# Autodesk Inventor assembly: Assembly1
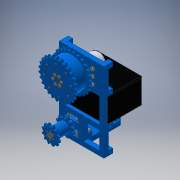
[picture p0: Inventor's stored thumbnail of the model, 180x180]
Saved by Autodesk Inventor 2016 (Build 200138000, 138)
## iProperties
Created: 2016-06-04
Part Number: Assembly1
Document SubType Name: Assembly
Designer: hesaon
Author: hesaon
## Documents named in this file (24)
- C:\Users\hesaon\Documents\Killer-Bot-2016\AutodeskWorkspace\robotparts revision 2\Assembly1.iam
- C:\Users\hesaon\Documents\Killer-Bot-2016\AutodeskWorkspace\robotparts revision 2\sideFrame.ipt
- C:\Users\hesaon\Documents\Killer-Bot-2016\AutodeskWorkspace\robotparts revision 2\motorHolder57mmVer2.ipt
- C:\Users\hesaon\Documents\Killer-Bot-2016\AutodeskWorkspace\robotparts revision 2\nut4mm.ipt
- C:\Users\hesaon\Documents\Killer-Bot-2016\AutodeskWorkspace\robotparts revision 2\screw18x4mm.ipt
- C:\Users\hesaon\Documents\Killer-Bot-2016\AutodeskWorkspace\robotparts revision 2\washer4mm.ipt
- C:\Users\hesaon\Documents\Killer-Bot-2016\AutodeskWorkspace\robotparts revision 2\37D mm metal gearmotor.ipt
- C:\Users\hesaon\Documents\Killer-Bot-2016\AutodeskWorkspace\robotparts revision 2\washer3mm.ipt
- C:\Users\hesaon\Documents\Killer-Bot-2016\AutodeskWorkspace\robotparts revision 2\screw12x3mm.ipt
- C:\Users\hesaon\Documents\Killer-Bot-2016\AutodeskWorkspace\robotparts revision 2\mountingHub6mm.ipt
- C:\Users\hesaon\Documents\Killer-Bot-2016\AutodeskWorkspace\robotparts revision 2\outerBigSprocket2.ipt
- C:\Users\hesaon\Documents\Killer-Bot-2016\AutodeskWorkspace\robotparts revision 2\sprocketsHolder.ipt
- C:\Users\hesaon\Documents\Killer-Bot-2016\AutodeskWorkspace\robotparts revision 2\BigSprocket2.ipt
- C:\Users\hesaon\Documents\Killer-Bot-2016\AutodeskWorkspace\robotparts revision 2\screwKa22x16.ipt
- C:\Users\hesaon\Documents\Killer-Bot-2016\AutodeskWorkspace\robotparts revision 2\battery.ipt
- C:\Users\hesaon\Documents\Killer-Bot-2016\AutodeskWorkspace\robotparts revision 2\backFrame.ipt
- C:\Users\hesaon\Documents\Killer-Bot-2016\AutodeskWorkspace\robotparts revision 2\screw27x4mm.ipt
- C:\Users\hesaon\Documents\Killer-Bot-2016\AutodeskWorkspace\robotparts revision 2\pin5x60.ipt
- C:\Users\hesaon\Documents\Killer-Bot-2016\AutodeskWorkspace\robotparts revision 2\smallSprocketFixture.ipt
- C:\Users\hesaon\Documents\Killer-Bot-2016\AutodeskWorkspace\robotparts revision 2\nut6mm.ipt
- C:\Users\hesaon\Documents\Killer-Bot-2016\AutodeskWorkspace\robotparts revision 2\washer6mm.ipt
- C:\Users\hesaon\Documents\Killer-Bot-2016\AutodeskWorkspace\robotparts revision 2\smallSprocketDistance.ipt
- C:\Users\hesaon\Documents\Killer-Bot-2016\AutodeskWorkspace\robotparts revision 2\smallSprocket.ipt
- C:\Users\hesaon\Documents\Killer-Bot-2016\AutodeskWorkspace\robotparts revision 2\smallSprocketHolder.ipt
## Components (105 placed, 22 different names)
1. sideFrame:1 — Insert:1, Insert:2, Insert:3, Insert:4, Insert:5, Insert:6, Insert:7, Insert:8, Flush:1, Mate:1, Mate:2, Insert:80, Insert:81, Insert:86, Insert:87, Insert:90, Insert:91
2. motorHolder57mmVer2:1 — Insert:1, Insert:2, Insert:9, Insert:10, Insert:11, Insert:12, Insert:13, Insert:14, Insert:27, Insert:28, Insert:29, Insert:30, Insert:31, Insert:32, Insert:33, Insert:34
3. nut4mm:1 — Insert:26
4. nut4mm:2 — Insert:21
5. nut4mm:3 — Insert:22
6. nut4mm:4 — Insert:23
7. nut4mm:5 — Insert:24
8. nut4mm:6 — Insert:25
9. screw18x4mm:1 — Insert:17
10. screw18x4mm:2 — Insert:19
11. screw18x4mm:3 — Insert:16
12. screw18x4mm:4 — Insert:15
13. screw18x4mm:5 — Insert:18
14. screw18x4mm:6 — Insert:20
15. washer4mm:1 — Insert:5, Insert:21
16. washer4mm:2 — Insert:8, Insert:24
17. washer4mm:3 — Insert:10, Insert:17
18. washer4mm:4 — Insert:9, Insert:15
19. washer4mm:5 — Insert:11, Insert:18
20. washer4mm:6 — Insert:12, Insert:19
21. washer4mm:7 — Insert:7, Insert:26
22. washer4mm:8 — Insert:13, Insert:16
23. washer4mm:9 — Insert:14, Insert:20
24. washer4mm:10 — Insert:4, Insert:23
25. washer4mm:11 — Insert:3, Insert:22
26. washer4mm:12 — Insert:6, Insert:25
27. 37D mm metal gearmotor:1 — Insert:27, Insert:28, Insert:41
28. washer3mm:1 — Insert:29, Insert:37
29. washer3mm:2 — Insert:30, Insert:36
30. washer3mm:3 — Insert:32, Insert:40
31. washer3mm:4 — Insert:31, Insert:35
32. washer3mm:5 — Insert:33, Insert:39
33. washer3mm:6 — Insert:34, Insert:38
34. screw12x3mm:1 — Insert:38
35. screw12x3mm:2 — Insert:35
36. screw12x3mm:3 — Insert:36
37. screw12x3mm:4 — Insert:37
38. screw12x3mm:5 — Insert:40
39. screw12x3mm:6 — Insert:39
40. mountingHub6mm:1 — Insert:41, Insert:42, Insert:43
41. Outer big sprocket:1 — Insert:42, Insert:43, Insert:44, Insert:45, Insert:48, Insert:49, Insert:50, Insert:51, Insert:52, Insert:53, Insert:54, Insert:55, Insert:64, Insert:65, Insert:66, Insert:67, Insert:68, Insert:69
42. sprocketsHolder:1 — Insert:44, Insert:45, Insert:46, Insert:47
43. Roller Chain Sprocket1:1 — Insert:46, Insert:47, Insert:56, Insert:57, Insert:58, Insert:59, Insert:60, Insert:61, Insert:62, Insert:63
44. screwKa22x16:1 — Insert:56
45. screwKa22x16:2 — Insert:57
46. screwKa22x16:3 — Insert:58
47. screwKa22x16:4 — Insert:59
48. screwKa22x16:5 — Insert:60
49. screwKa22x16:6 — Insert:61
50. screwKa22x16:7 — Insert:63
51. screwKa22x16:8 — Insert:62
52. screwKa22x16:9 — Insert:48
53. screwKa22x16:10 — Insert:49
54. screwKa22x16:11 — Insert:50
55. screwKa22x16:12 — Insert:51
56. screwKa22x16:13 — Insert:52
57. screwKa22x16:14 — Insert:53
58. screwKa22x16:15 — Insert:54
59. screwKa22x16:16 — Insert:55
60. washer3mm:7 — Insert:64, Insert:70
61. washer3mm:8 — Insert:65, Insert:74
62. washer3mm:9 — Insert:66, Insert:75
63. washer3mm:10 — Insert:67, Insert:73
64. washer3mm:11 — Insert:68, Insert:72
65. washer3mm:12 — Insert:69, Insert:71
66. screw12x3mm:7 — Insert:70
67. screw12x3mm:8 — Insert:71
68. screw12x3mm:9 — Insert:72
69. screw12x3mm:10 — Insert:73
70. screw12x3mm:11 — Insert:74
71. screw12x3mm:12 — Insert:75
72. battery:1 — Flush:1, Mate:1, Mate:2
73. backFrame:1 — Insert:86, Insert:87, Insert:88, Insert:89
74. nut4mm:7 — Insert:85
75. nut4mm:8 — Insert:84
76. washer4mm:13 — Insert:82, Insert:89
77. washer4mm:14 — Insert:83, Insert:88
78. washer4mm:15 — Insert:80, Insert:85
79. washer4mm:16 — Insert:81, Insert:84
80. screw27x4mm:1 — Insert:83
81. screw27x4mm:2 — Insert:82
82. pin5x60:1 — Insert:91, Cylindrical:2
83. pin5x60:2 — Insert:90, Cylindrical:1
84. smallSprocketFixture:1 — Cylindrical:1, Cylindrical:2, Insert:92, Angle:1, Insert:94
85. nut6mm:1 — Insert:92, Angle:1, Insert:93
86. washer6mm:1 — Insert:93, Insert:95
87. washer6mm:2 — Insert:94
88. smallSprocketDistance:1 — Insert:95, Insert:96
89. washer6mm:3 — Insert:96, Insert:97
90. Roller Chain Sprocket1:2 — Insert:100, Insert:101, Insert:102, Insert:103, Insert:104, Insert:105, Insert:106, Insert:107, Insert:114
91. Roller Chain Sprocket1:3 — Insert:97, Insert:98, Insert:99, Insert:108, Insert:109, Insert:110, Insert:111, Insert:112, Insert:113
92. smallSprocketHolder:1 — Insert:98, Insert:99, Insert:100, Insert:101
93. screwKa22x16:17 — Insert:111
94. screwKa22x16:18 — Insert:104
95. screwKa22x16:19 — Insert:105
96. screwKa22x16:20 — Insert:106
97. screwKa22x16:21 — Insert:107
98. screwKa22x16:22 — Insert:109
99. screwKa22x16:23 — Insert:110
100. screwKa22x16:24 — Insert:112
101. screwKa22x16:25 — Insert:113
102. screwKa22x16:26 — Insert:108
103. screwKa22x16:27 — Insert:103
104. screwKa22x16:28 — Insert:102
105. washer6mm:4 — Insert:114
## Relationships (116: Insert 110, Mate 2, CylindricalJoint 2, Flush 1, Angle 1)
- Insert:1: sideFrame:1 ↔ motorHolder57mmVer2:1
- Insert:2: sideFrame:1 ↔ motorHolder57mmVer2:1
- Insert:3: sideFrame:1 ↔ washer4mm:11
- Insert:4: sideFrame:1 ↔ washer4mm:10
- Insert:5: sideFrame:1 ↔ washer4mm:1
- Insert:6: sideFrame:1 ↔ washer4mm:12
- Insert:7: sideFrame:1 ↔ washer4mm:7
- Insert:8: sideFrame:1 ↔ washer4mm:2
- Insert:9: motorHolder57mmVer2:1 ↔ washer4mm:4
- Insert:10: motorHolder57mmVer2:1 ↔ washer4mm:3
- Insert:11: motorHolder57mmVer2:1 ↔ washer4mm:5
- Insert:12: motorHolder57mmVer2:1 ↔ washer4mm:6
- Insert:13: motorHolder57mmVer2:1 ↔ washer4mm:8
- Insert:14: motorHolder57mmVer2:1 ↔ washer4mm:9
- Insert:15: screw18x4mm:4 ↔ washer4mm:4
- Insert:16: screw18x4mm:3 ↔ washer4mm:8
- Insert:17: screw18x4mm:1 ↔ washer4mm:3
- Insert:18: screw18x4mm:5 ↔ washer4mm:5
- Insert:19: screw18x4mm:2 ↔ washer4mm:6
- Insert:20: screw18x4mm:6 ↔ washer4mm:9
- Insert:21: nut4mm:2 ↔ washer4mm:1
- Insert:22: nut4mm:3 ↔ washer4mm:11
- Insert:23: nut4mm:4 ↔ washer4mm:10
- Insert:24: nut4mm:5 ↔ washer4mm:2
- Insert:25: nut4mm:6 ↔ washer4mm:12
- Insert:26: nut4mm:1 ↔ washer4mm:7
- Insert:27: motorHolder57mmVer2:1 ↔ 37D mm metal gearmotor:1
- Insert:28: motorHolder57mmVer2:1 ↔ 37D mm metal gearmotor:1
- Insert:29: motorHolder57mmVer2:1 ↔ washer3mm:1
- Insert:30: motorHolder57mmVer2:1 ↔ washer3mm:2
- Insert:31: motorHolder57mmVer2:1 ↔ washer3mm:4
- Insert:32: motorHolder57mmVer2:1 ↔ washer3mm:3
- Insert:33: motorHolder57mmVer2:1 ↔ washer3mm:5
- Insert:34: motorHolder57mmVer2:1 ↔ washer3mm:6
- Insert:35: washer3mm:4 ↔ screw12x3mm:2
- Insert:36: washer3mm:2 ↔ screw12x3mm:3
- Insert:37: washer3mm:1 ↔ screw12x3mm:4
- Insert:38: washer3mm:6 ↔ screw12x3mm:1
- Insert:39: washer3mm:5 ↔ screw12x3mm:6
- Insert:40: washer3mm:3 ↔ screw12x3mm:5
- Insert:41: 37D mm metal gearmotor:1 ↔ mountingHub6mm:1
- Insert:42: mountingHub6mm:1 ↔ Outer big sprocket:1
- Insert:43: mountingHub6mm:1 ↔ Outer big sprocket:1
- Insert:44: Outer big sprocket:1 ↔ sprocketsHolder:1
- Insert:45: Outer big sprocket:1 ↔ sprocketsHolder:1
- Insert:46: sprocketsHolder:1 ↔ Roller Chain Sprocket1:1
- Insert:47: sprocketsHolder:1 ↔ Roller Chain Sprocket1:1
- Insert:48: Outer big sprocket:1 ↔ screwKa22x16:9
- Insert:49: Outer big sprocket:1 ↔ screwKa22x16:10
- Insert:50: Outer big sprocket:1 ↔ screwKa22x16:11
- Insert:51: Outer big sprocket:1 ↔ screwKa22x16:12
- Insert:52: Outer big sprocket:1 ↔ screwKa22x16:13
- Insert:53: Outer big sprocket:1 ↔ screwKa22x16:14
- Insert:54: Outer big sprocket:1 ↔ screwKa22x16:15
- Insert:55: Outer big sprocket:1 ↔ screwKa22x16:16
- Insert:56: Roller Chain Sprocket1:1 ↔ screwKa22x16:1
- Insert:57: Roller Chain Sprocket1:1 ↔ screwKa22x16:2
- Insert:58: Roller Chain Sprocket1:1 ↔ screwKa22x16:3
- Insert:59: Roller Chain Sprocket1:1 ↔ screwKa22x16:4
- Insert:60: Roller Chain Sprocket1:1 ↔ screwKa22x16:5
- Insert:61: Roller Chain Sprocket1:1 ↔ screwKa22x16:6
- Insert:62: Roller Chain Sprocket1:1 ↔ screwKa22x16:8
- Insert:63: Roller Chain Sprocket1:1 ↔ screwKa22x16:7
- Insert:64: Outer big sprocket:1 ↔ washer3mm:7
- Insert:65: Outer big sprocket:1 ↔ washer3mm:8
- Insert:66: Outer big sprocket:1 ↔ washer3mm:9
- Insert:67: Outer big sprocket:1 ↔ washer3mm:10
- Insert:68: Outer big sprocket:1 ↔ washer3mm:11
- Insert:69: Outer big sprocket:1 ↔ washer3mm:12
- Insert:70: washer3mm:7 ↔ screw12x3mm:7
- Insert:71: washer3mm:12 ↔ screw12x3mm:8
- Insert:72: washer3mm:11 ↔ screw12x3mm:9
- Insert:73: washer3mm:10 ↔ screw12x3mm:10
- Insert:74: washer3mm:8 ↔ screw12x3mm:11
- Insert:75: washer3mm:9 ↔ screw12x3mm:12
- Flush:1: sideFrame:1 ↔ battery:1
- Mate:1: sideFrame:1 ↔ battery:1
- Mate:2: sideFrame:1 ↔ battery:1
- Insert:80: sideFrame:1 ↔ washer4mm:15
- Insert:81: sideFrame:1 ↔ washer4mm:16
- Insert:82: washer4mm:13 ↔ screw27x4mm:2
- Insert:83: washer4mm:14 ↔ screw27x4mm:1
- Insert:84: nut4mm:8 ↔ washer4mm:16
- Insert:85: nut4mm:7 ↔ washer4mm:15
- Insert:86: sideFrame:1 ↔ backFrame:1
- Insert:87: sideFrame:1 ↔ backFrame:1
- Insert:88: backFrame:1 ↔ washer4mm:14
- Insert:89: backFrame:1 ↔ washer4mm:13
- Insert:90: sideFrame:1 ↔ pin5x60:2
- Insert:91: sideFrame:1 ↔ pin5x60:1
- Cylindrical:1: pin5x60:2 ↔ smallSprocketFixture:1
- Cylindrical:2: pin5x60:1 ↔ smallSprocketFixture:1
- Insert:92: smallSprocketFixture:1 ↔ nut6mm:1
- Angle:1 (0 deg): smallSprocketFixture:1 ↔ nut6mm:1
- Insert:93: nut6mm:1 ↔ washer6mm:1
- Insert:94: smallSprocketFixture:1 ↔ washer6mm:2
- Insert:95: washer6mm:1 ↔ smallSprocketDistance:1
- Insert:96: smallSprocketDistance:1 ↔ washer6mm:3
- Insert:97: washer6mm:3 ↔ Roller Chain Sprocket1:3
- Insert:98: Roller Chain Sprocket1:3 ↔ smallSprocketHolder:1
- Insert:99: Roller Chain Sprocket1:3 ↔ smallSprocketHolder:1
- Insert:100: Roller Chain Sprocket1:2 ↔ smallSprocketHolder:1
- Insert:101: Roller Chain Sprocket1:2 ↔ smallSprocketHolder:1
- Insert:102: Roller Chain Sprocket1:2 ↔ screwKa22x16:28
- Insert:103: Roller Chain Sprocket1:2 ↔ screwKa22x16:27
- Insert:104: Roller Chain Sprocket1:2 ↔ screwKa22x16:18
- Insert:105: Roller Chain Sprocket1:2 ↔ screwKa22x16:19
- Insert:106: Roller Chain Sprocket1:2 ↔ screwKa22x16:20
- Insert:107: Roller Chain Sprocket1:2 ↔ screwKa22x16:21
- Insert:108: Roller Chain Sprocket1:3 ↔ screwKa22x16:26
- Insert:109: Roller Chain Sprocket1:3 ↔ screwKa22x16:22
- Insert:110: Roller Chain Sprocket1:3 ↔ screwKa22x16:23
- Insert:111: Roller Chain Sprocket1:3 ↔ screwKa22x16:17
- Insert:112: Roller Chain Sprocket1:3 ↔ screwKa22x16:24
- Insert:113: Roller Chain Sprocket1:3 ↔ screwKa22x16:25
- Insert:114: Roller Chain Sprocket1:2 ↔ washer6mm:4
